# Autodesk Inventor assembly: Assembly1_MIR1
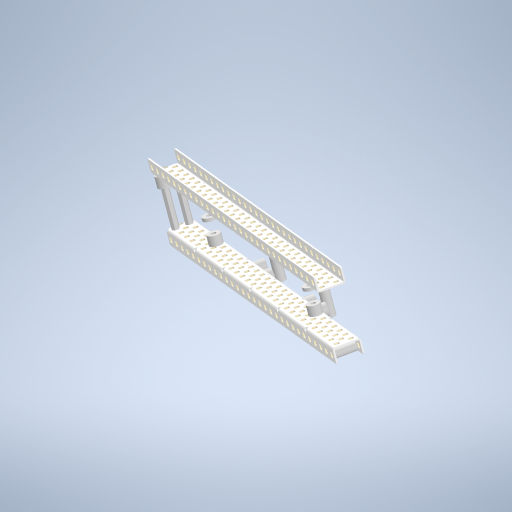
[picture p0: Inventor's stored thumbnail of the model, 512x512]
Saved by Autodesk Inventor 2024 (Build 280153000, 153)
## iProperties
Created: 2023-09-19
Part Number: Assembly1_MIR1
Document SubType Name: Assembly
Designer: Robodox
Author: Robodox
## Documents named in this file (9)
- C:\Users\Robodox\Documents\GitHub\VEXCAD\Assembly1_MIR1.iam
- C:\Users\Robodox\Documents\GitHub\VEXCAD\Part1_MIR1.ipt
- C:\Users\Robodox\Documents\GitHub\VEXCAD\Part2_MIR2.ipt
- C:\Users\Robodox\Documents\GitHub\VEXCAD\Part3_MIR1.ipt
- C:\Users\Robodox\Documents\GitHub\VEXCAD\Part5_MIR1.ipt
- C:\Users\Robodox\Documents\GitHub\VEXCAD\part8_MIR1.ipt
- C:\Users\Robodox\Documents\GitHub\VEXCAD\Part4.ipt
- C:\Users\Robodox\Documents\GitHub\VEXCAD\washer.ipt
- C:\Users\Robodox\Documents\GitHub\VEX-CAD-Inventor\Structure\C Channel\Aluminum 1x2x1\Alu C 1x2x1x30.ipt
## Components (32 placed, 8 different names)
1. Part2_MIR2:3 — Mate:29, Mate:14, Mate:28, Mate:13
2. Part1_MIR1:5 — Mate:29, Mate:14, Mate:114
3. Part1_MIR1:6 — Mate:28, Mate:13, Mate:111, Mate:112
4. Part3_MIR1:1 — Mate:113, Mate:114
5. Part3_MIR1:2 — Mate:115
6. Part3_MIR1:3 — Mate:118, Mate:119
7. Part3_MIR1:4 — Mate:120, Mate:121
8. Part5_MIR1:1 — Mate:52, Mate:47
9. Part5_MIR1:2 — Mate:49, Mate:48
10. Part5_MIR1:3 — Mate:52, Mate:47
11. Part5_MIR1:4 — Mate:49, Mate:48
12. part8_MIR1:1
13. part8_MIR1:2
14. part8_MIR1:3
15. Part3_MIR1:5
16. Part3_MIR1:6
17. Part1_MIR1:2 — Mate:6, Mate:3, Mate:103
18. Part2_MIR2:1 — Mate:5, Mate:4, Mate:6, Mate:3, Mate:102
19. Part1_MIR1:1 — Mate:5, Mate:4
20. Part1_MIR1:4 — Mate:30, Mate:8, Mate:116, Mate:117
21. Part2_MIR2:2 — Mate:30, Mate:10, Mate:9, Mate:8
22. Part1_MIR1:3 — Mate:10, Mate:9
23. Part2_MIR2:4 — Mate:109, Mate:108
24. Part1_MIR1:7 — Mate:109, Mate:108, Mate:122, Mate:123
25. Part4:1 — Mate:89, Mate:90
26. Part3_MIR1:7 — Mate:83, Mate:86, Mate:88
27. Part3_MIR1:8 — Mate:84, Mate:85, Mate:90, Mate:100
28. Part4:2 — Mate:87, Mate:88, Mate:110
29. washer:1 — Mate:84, Mate:85, Mate:89
30. washer:2 — Mate:83, Mate:86, Mate:87
31. Alu C 1x2x1x30:1 — Mate:100, Flush:1, Flush:2, Mate:109
32. Alu C 1x2x1x30:2 — Flush:1, Flush:2, Mate:102, Mate:103, Mate:109, Mate:110, Mate:111, Mate:112, Mate:113, Mate:115, Mate:116, Mate:117, Mate:118, Mate:119, Mate:120, Mate:121, Mate:122, Mate:123
## Relationships (46: Mate 44, Flush 2)
- Mate:5: Part2_MIR2:1 ↔ Part1_MIR1:1
- Mate:4: Part2_MIR2:1 ↔ Part1_MIR1:1
- Mate:6: Part1_MIR1:2 ↔ Part2_MIR2:1
- Mate:3: Part1_MIR1:2 ↔ Part2_MIR2:1
- Mate:30: Part1_MIR1:4 ↔ Part2_MIR2:2
- Mate:10: Part2_MIR2:2 ↔ Part1_MIR1:3
- Mate:9: Part2_MIR2:2 ↔ Part1_MIR1:3
- Mate:8: Part1_MIR1:4 ↔ Part2_MIR2:2
- Mate:29: Part2_MIR2:3 ↔ Part1_MIR1:5
- Mate:14: Part2_MIR2:3 ↔ Part1_MIR1:5
- Mate:28: Part2_MIR2:3 ↔ Part1_MIR1:6
- Mate:13: Part2_MIR2:3 ↔ Part1_MIR1:6
- Mate:52: Part5_MIR1:1 ↔ Part5_MIR1:3
- Mate:47: Part5_MIR1:1 ↔ Part5_MIR1:3
- Mate:49: Part5_MIR1:2 ↔ Part5_MIR1:4
- Mate:48: Part5_MIR1:2 ↔ Part5_MIR1:4
- Mate:109: Part2_MIR2:4 ↔ Part1_MIR1:7
- Mate:108: Part2_MIR2:4 ↔ Part1_MIR1:7
- Mate:83: Part3_MIR1:7 ↔ washer:2
- Mate:84: Part3_MIR1:8 ↔ washer:1
- Mate:85: Part3_MIR1:8 ↔ washer:1
- Mate:86: Part3_MIR1:7 ↔ washer:2
- Mate:87: Part4:2 ↔ washer:2
- Mate:88: Part3_MIR1:7 ↔ Part4:2
- Mate:89: Part4:1 ↔ washer:1
- Mate:90: Part4:1 ↔ Part3_MIR1:8
- Mate:100: Part3_MIR1:8 ↔ Alu C 1x2x1x30:1
- Flush:1: Alu C 1x2x1x30:1 ↔ Alu C 1x2x1x30:2
- Flush:2: Alu C 1x2x1x30:1 ↔ Alu C 1x2x1x30:2
- Mate:102: Part2_MIR2:1 ↔ Alu C 1x2x1x30:2
- Mate:103: Part1_MIR1:2 ↔ Alu C 1x2x1x30:2
- Mate:109 (64.77 mm): Alu C 1x2x1x30:1 ↔ Alu C 1x2x1x30:2
- Mate:110: Part4:2 ↔ Alu C 1x2x1x30:2
- Mate:111: Part1_MIR1:6 ↔ Alu C 1x2x1x30:2
- Mate:112: Part1_MIR1:6 ↔ Alu C 1x2x1x30:2
- Mate:113: Part3_MIR1:1 ↔ Alu C 1x2x1x30:2
- Mate:114: Part1_MIR1:5 ↔ Part3_MIR1:1
- Mate:115: Part3_MIR1:2 ↔ Alu C 1x2x1x30:2
- Mate:116: Part1_MIR1:4 ↔ Alu C 1x2x1x30:2
- Mate:117: Part1_MIR1:4 ↔ Alu C 1x2x1x30:2
- Mate:118: Part3_MIR1:3 ↔ Alu C 1x2x1x30:2
- Mate:119: Part3_MIR1:3 ↔ Alu C 1x2x1x30:2
- Mate:120: Part3_MIR1:4 ↔ Alu C 1x2x1x30:2
- Mate:121: Part3_MIR1:4 ↔ Alu C 1x2x1x30:2
- Mate:122: Part1_MIR1:7 ↔ Alu C 1x2x1x30:2
- Mate:123: Part1_MIR1:7 ↔ Alu C 1x2x1x30:2
